# Autodesk Inventor assembly: Assembly2
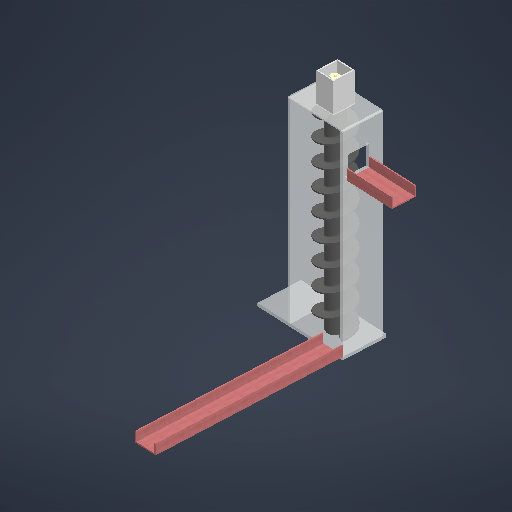
[picture p0: Inventor's stored thumbnail of the model, 512x512]
Saved by Autodesk Inventor 2026.2 (Build 302298000, 298)
## iProperties
Created: 2026-03-02
Part Number: Assembly2
Document SubType Name: Assembly
Designer: shahd
Author: shahd
## Documents named in this file (10)
- C:\Users\danda\BOM-project\Project\CAD\Lifting\Lifting\liftingAssembly2.iam
- C:\Users\danda\BOM-project\Project\CAD\Lifting\Lifting\Part3.ipt
- C:\Users\danda\BOM-project\Project\CAD\Lifting\Lifting\Part4.ipt
- C:\Users\danda\BOM-project\Project\CAD\Lifting\Lifting\Lifting Mechanism.ipt
- C:\Users\danda\BOM-project\Project\CAD\Lifting\Lifting\base.ipt
- C:\Users\danda\BOM-project\Project\CAD\Lifting\Lifting\slide1.ipt
- C:\Users\danda\BOM-project\Project\CAD\Lifting\Lifting\slide2.ipt
- C:\Users\danda\BOM-project\Project\CAD\Lifting\Lifting\partttt.ipt
- C:\Users\danda\BOM-project\Project\CAD\Lifting\Lifting\motor box.ipt
- C:\Users\danda\BOM-project\Project\CAD\Lifting\Lifting\Motor DC 16mm.ipt
## Components (12 placed, 9 different names)
1. Part3:1 — Mate:1, Mate:4, Flush:2, Mate:5, Mate:18, Flush:10
2. Part4:1 — Mate:1, Mate:4, Flush:2, Flush:3, Flush:4, Mate:9, Flush:5, Flush:6, Flush:7, Mate:21, Mate:22, Mate:23, Mate:24, Mate:25, Mate:27, Mate:28
3. Lifting Mechanism:1 — Mate:8, Mate:26
4. base:1 — Mate:5, Mate:8, Flush:8, Mate:10, Mate:11, Mate:18, Flush:10
5. slide1:1 — Mate:10, Mate:11, Flush:17
6. slide2:1 — Mate:13, Mate:14, Mate:15, Mate:16, Flush:9, Mate:17
7. partttt:1 — Flush:3, Flush:4, Mate:9, Flush:5, Flush:6, Flush:7, Flush:8, Mate:13, Mate:14, Mate:15, Mate:16, Flush:9, Mate:17, Flush:17
8. motor box:1 — Mate:22, Mate:23, Flush:11, Flush:12
9. motor box:2 — Mate:21, Flush:13, Flush:14, Flush:15, Flush:16
10. motor box:4 — Mate:25, Flush:12, Flush:14, Flush:15
11. motor box:5 — Mate:24, Flush:11, Flush:13, Flush:16
12. Motor DC 16mm:1 — Mate:26, Mate:27, Mate:28
## Relationships (37: Mate 21, Flush 16)
- Mate:1: Part3:1 ↔ Part4:1
- Mate:4: Part3:1 ↔ Part4:1
- Flush:2: Part3:1 ↔ Part4:1
- Mate:5: Part3:1 ↔ base:1
- Mate:8: Lifting Mechanism:1 ↔ base:1
- Flush:3: Part4:1 ↔ partttt:1
- Flush:4: Part4:1 ↔ partttt:1
- Mate:9: Part4:1 ↔ partttt:1
- Flush:5: Part4:1 ↔ partttt:1
- Flush:6: Part4:1 ↔ partttt:1
- Flush:7: Part4:1 ↔ partttt:1
- Flush:8: base:1 ↔ partttt:1
- Mate:10: base:1 ↔ slide1:1
- Mate:11: base:1 ↔ slide1:1
- Mate:13: slide2:1 ↔ partttt:1
- Mate:14: slide2:1 ↔ partttt:1
- Mate:15: slide2:1 ↔ partttt:1
- Mate:16: slide2:1 ↔ partttt:1
- Flush:9: slide2:1 ↔ partttt:1
- Mate:17: slide2:1 ↔ partttt:1
- Mate:18: Part3:1 ↔ base:1
- Flush:10: Part3:1 ↔ base:1
- Mate:21: Part4:1 ↔ motor box:2
- Mate:22: Part4:1 ↔ motor box:1
- Mate:23: Part4:1 ↔ motor box:1
- Mate:24: Part4:1 ↔ motor box:5
- Mate:25: Part4:1 ↔ motor box:4
- Flush:11: motor box:1 ↔ motor box:5
- Flush:12: motor box:1 ↔ motor box:4
- Flush:13: motor box:2 ↔ motor box:5
- Flush:14: motor box:2 ↔ motor box:4
- Flush:15: motor box:2 ↔ motor box:4
- Flush:16: motor box:2 ↔ motor box:5
- Mate:26: Lifting Mechanism:1 ↔ Motor DC 16mm:1
- Mate:27: Part4:1 ↔ Motor DC 16mm:1
- Mate:28: Part4:1 ↔ Motor DC 16mm:1
- Flush:17: slide1:1 ↔ partttt:1
